# Autodesk Inventor assembly: Z Axis
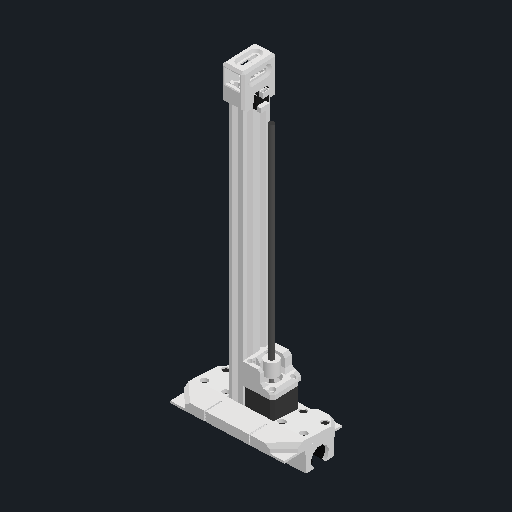
[picture p0: Inventor's stored thumbnail of the model, 512x512]
Saved by Autodesk Inventor 2026 (Build 300175000, 175)
## iProperties
Created: 2025-01-21
Part Number: Z Axis
Document SubType Name: Assembly
Designer: jerem
Author: jerem
## Documents named in this file (13)
- C:\Users\jerem\Documents\GitHub\Perovskite-Automated-Synthesis-System\CAD\Gantry\Z Axis\Z Axis.iam
- C:\Users\jerem\Documents\GitHub\Perovskite-Automated-Synthesis-System\CAD\Non 3D Printed Parts\Extrusion\V Extrustion 40x400mm.ipt
- C:\Users\jerem\Documents\GitHub\Perovskite-Automated-Synthesis-System\CAD\Non 3D Printed Parts\Screws\M5x12.ipt
- C:\Users\jerem\Documents\GitHub\Perovskite-Automated-Synthesis-System\CAD\Non 3D Printed Parts\Motors and Servos\NEMA17 Stepper Motor.ipt
- C:\Users\jerem\Documents\GitHub\Perovskite-Automated-Synthesis-System\CAD\Non 3D Printed Parts\Threaded Rod 300mm.ipt
- C:\Users\jerem\Documents\GitHub\Perovskite-Automated-Synthesis-System\CAD\Non 3D Printed Parts\Rod Coupler.ipt
- C:\Users\jerem\Documents\GitHub\Perovskite-Automated-Synthesis-System\CAD\Non 3D Printed Parts\Nuts\M4 T-Slot Nut.ipt
- C:\Users\jerem\Documents\GitHub\Perovskite-Automated-Synthesis-System\CAD\Gantry\Z Axis\Z Axis Motor Mount.ipt
- C:\Users\jerem\Documents\GitHub\Perovskite-Automated-Synthesis-System\CAD\Non 3D Printed Parts\Linear Rails\Linear Rail Slider Block.ipt
- C:\Users\jerem\Documents\GitHub\Perovskite-Automated-Synthesis-System\CAD\Non 3D Printed Parts\X Axis Base Plate Accurate.ipt
- C:\Users\jerem\Documents\GitHub\Perovskite-Automated-Synthesis-System\CAD\Gantry\X Axis\X-Base Cover.ipt
- C:\Users\jerem\Documents\GitHub\Perovskite-Automated-Synthesis-System\CAD\Gantry\Z Axis\Z Axis Cap.ipt
- C:\Users\jerem\Documents\GitHub\Perovskite-Automated-Synthesis-System\CAD\Non 3D Printed Parts\Limit Switch.ipt
## Components (21 placed, 12 different names)
1. V Extrustion 40x400mm:1 — Mate:54, Mate:25, Mate:30, Angle:2, Angle:3, Mate:32, Flush:1, Mate:53, Mate:55, Mate:75, Mate:76, Flush:2
2. M5x12:1 — Mate:47, Mate:68
3. M5x12:2 — Mate:49, Mate:51, Mate:71
4. M5x12:3 — Mate:59, Mate:66
5. M5x12:4 — Mate:58, Mate:65
6. M5x12:5 — Mate:48, Mate:50, Mate:69
7. M5x12:7 — Mate:46, Mate:70
8. NEMA17 Stepper Motor:1 — Mate:25, Mate:33, Mate:34, Mate:35, Flush:1, Mate:63
9. Threaded Rod 300mm:1
10. Rod Coupler:1
11. M4 T-Slot Nut:1 — Mate:30, Angle:2, Mate:37
12. M4 T-Slot Nut:2 — Angle:3, Mate:32, Mate:36
13. Z Axis Motor Mount:1 — Mate:33, Mate:34, Mate:35, Mate:36, Mate:37
14. Linear Rail Slider Block:2 — Mate:46, Mate:47, Mate:50, Mate:51, Mate:52
15. X Axis Base Plate Accurate:1 — Mate:48, Mate:49, Mate:52, Mate:53, Mate:54, Mate:55, Mate:56, Mate:57, Mate:58, Mate:59, Mate:60, Mate:61, Mate:62, Mate:63, Mate:64, Mate:65, Mate:66, Mate:67, Mate:68, Mate:69, Mate:70, Mate:71, Mate:72, Mate:73, Mate:74
16. Linear Rail Slider Block:3 — Mate:56, Mate:57, Mate:60
17. M5x12:8 — Mate:62, Mate:64
18. M5x12:9 — Mate:61, Mate:67
19. X-Base Cover:1 — Mate:72, Mate:73, Mate:74
20. Z Axis Cap:1 — Mate:75, Mate:76, Flush:2, Mate:77, Mate:78, Mate:79
21. Limit Switch:1 — Mate:77, Mate:78, Mate:79
## Relationships (50: Mate 46, Angle 2, Flush 2)
- [Mate]: NEMA17 Stepper Motor:1 ↔ Rod Coupler:1
- [Mate]: Threaded Rod 300mm:1 ↔ Rod Coupler:1
- [Mate] (-8 mm): NEMA17 Stepper Motor:1 ↔ Rod Coupler:1
- [Mate] (-8 mm): Threaded Rod 300mm:1 ↔ Rod Coupler:1
- Mate:54: V Extrustion 40x400mm:1 ↔ X Axis Base Plate Accurate:1
- Mate:25: V Extrustion 40x400mm:1 ↔ NEMA17 Stepper Motor:1
- Mate:30: V Extrustion 40x400mm:1 ↔ M4 T-Slot Nut:1
- Angle:2 (0 deg): V Extrustion 40x400mm:1 ↔ M4 T-Slot Nut:1
- Angle:3 (0 deg): V Extrustion 40x400mm:1 ↔ M4 T-Slot Nut:2
- Mate:32: V Extrustion 40x400mm:1 ↔ M4 T-Slot Nut:2
- Mate:33: NEMA17 Stepper Motor:1 ↔ Z Axis Motor Mount:1
- Mate:34: NEMA17 Stepper Motor:1 ↔ Z Axis Motor Mount:1
- Mate:35: NEMA17 Stepper Motor:1 ↔ Z Axis Motor Mount:1
- Mate:36: M4 T-Slot Nut:2 ↔ Z Axis Motor Mount:1
- Mate:37: M4 T-Slot Nut:1 ↔ Z Axis Motor Mount:1
- Flush:1: V Extrustion 40x400mm:1 ↔ NEMA17 Stepper Motor:1
- Mate:46: M5x12:7 ↔ Linear Rail Slider Block:2
- Mate:47: M5x12:1 ↔ Linear Rail Slider Block:2
- Mate:48: M5x12:5 ↔ X Axis Base Plate Accurate:1
- Mate:49: M5x12:2 ↔ X Axis Base Plate Accurate:1
- Mate:50: M5x12:5 ↔ Linear Rail Slider Block:2
- Mate:51: M5x12:2 ↔ Linear Rail Slider Block:2
- Mate:52: Linear Rail Slider Block:2 ↔ X Axis Base Plate Accurate:1
- Mate:53: V Extrustion 40x400mm:1 ↔ X Axis Base Plate Accurate:1
- Mate:55: V Extrustion 40x400mm:1 ↔ X Axis Base Plate Accurate:1
- Mate:56: X Axis Base Plate Accurate:1 ↔ Linear Rail Slider Block:3
- Mate:57: X Axis Base Plate Accurate:1 ↔ Linear Rail Slider Block:3
- Mate:58: M5x12:4 ↔ X Axis Base Plate Accurate:1
- Mate:59: M5x12:3 ↔ X Axis Base Plate Accurate:1
- Mate:60: X Axis Base Plate Accurate:1 ↔ Linear Rail Slider Block:3
- Mate:61: X Axis Base Plate Accurate:1 ↔ M5x12:9
- Mate:62: X Axis Base Plate Accurate:1 ↔ M5x12:8
- Mate:63: NEMA17 Stepper Motor:1 ↔ X Axis Base Plate Accurate:1
- Mate:64: X Axis Base Plate Accurate:1 ↔ M5x12:8
- Mate:65: M5x12:4 ↔ X Axis Base Plate Accurate:1
- Mate:66: M5x12:3 ↔ X Axis Base Plate Accurate:1
- Mate:67: X Axis Base Plate Accurate:1 ↔ M5x12:9
- Mate:68: M5x12:1 ↔ X Axis Base Plate Accurate:1
- Mate:69: M5x12:5 ↔ X Axis Base Plate Accurate:1
- Mate:70: M5x12:7 ↔ X Axis Base Plate Accurate:1
- Mate:71: M5x12:2 ↔ X Axis Base Plate Accurate:1
- Mate:72: X Axis Base Plate Accurate:1 ↔ X-Base Cover:1
- Mate:73: X Axis Base Plate Accurate:1 ↔ X-Base Cover:1
- Mate:74: X Axis Base Plate Accurate:1 ↔ X-Base Cover:1
- Mate:75: V Extrustion 40x400mm:1 ↔ Z Axis Cap:1
- Mate:76: V Extrustion 40x400mm:1 ↔ Z Axis Cap:1
- Flush:2: V Extrustion 40x400mm:1 ↔ Z Axis Cap:1
- Mate:77: Z Axis Cap:1 ↔ Limit Switch:1
- Mate:78: Z Axis Cap:1 ↔ Limit Switch:1
- Mate:79: Z Axis Cap:1 ↔ Limit Switch:1
